# Autodesk Inventor assembly: Assembly
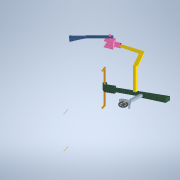
[picture p0: Inventor's stored thumbnail of the model, 180x180]
Saved by Autodesk Inventor 2021 (Build 250183000, 183)
## iProperties
Created: 2021-05-09
Part Number: Assembly
Document SubType Name: Assembly
Designer: Alsayaary
Author: Abdulrahman
## Documents named in this file (9)
- \\userAB\A\alsa0009\Desktop\seccuring mechanism\Assembly.iam
- \\userAB\A\alsa0009\Desktop\Securing mechanism paramatrised711\grip - C1-1.ipt
- \\userAB\A\alsa0009\Desktop\Securing mechanism paramatrised711\grip - C2-1.ipt
- \\userAB\A\alsa0009\Desktop\Securing mechanism paramatrised711\grip - C4-1.ipt
- \\userAB\A\alsa0009\Desktop\Securing mechanism paramatrised711\pin-1.ipt
- \\userAB\A\alsa0009\Desktop\Cad\sweep.ipt
- \\userAB\A\alsa0009\Desktop\Cad\wheel2.ipt
- \\userAB\A\alsa0009\Desktop\Securing mechanism paramatrised711\grip - Copy1-1.ipt
- \\userAB\A\alsa0009\Desktop\Cad\handle.ipt
## Components (8 placed, 8 different names)
1. grip - C1-1:1 — Mate:1, Mate:2, Flush:1, Mate:3, Flush:2, Mate:4, Mate:5, Mate:7, Mate:8, Flush:3, Mate:14, Transitional:1
2. grip - C2-1:1 — Mate:5, Mate:7, Mate:8, Flush:3, Mate:16, Mate:17, Mate:19
3. grip - C4-1:1 — Mate:3, Flush:2, Mate:4, Mate:15
4. sweep:1 — Mate:9, Mate:10, Transitional:1
5. wheel2:1 — Mate:15, Angle:3
6. pin-1:2 — Mate:16, Mate:18
7. grip - Copy1-1:1 — Mate:17, Mate:18, Mate:19, Mate:20, Mate:21
8. handle:1 — Mate:20, Mate:21
## Relationships (28: Mate 19, Flush 4, Angle 3, Symmetry 1, Transitional 1)
- Mate:1: grip - C1-1:1
- Mate:2: grip - C1-1:1
- Flush:1: grip - C1-1:1
- Mate:3: grip - C1-1:1 ↔ grip - C4-1:1
- Flush:2 (6.27 mm): grip - C1-1:1 ↔ grip - C4-1:1
- Mate:4 (231.798 mm): grip - C1-1:1 ↔ grip - C4-1:1
- Mate:5: grip - C1-1:1 ↔ grip - C2-1:1
- Mate:7: grip - C1-1:1 ↔ grip - C2-1:1
- Mate:8 (313.691 mm): grip - C1-1:1 ↔ grip - C2-1:1
- Flush:3: grip - C1-1:1 ↔ grip - C2-1:1
- Mate:9: sweep:1
- Mate:10: sweep:1
- Mate:11
- Angle:1 (0 deg)
- Mate:12
- Angle:2 (0 deg)
- Symmetry:1
- Flush:4
- Mate:14: grip - C1-1:1
- Mate:15: grip - C4-1:1 ↔ wheel2:1
- Angle:3 (0 deg): wheel2:1
- Mate:16: grip - C2-1:1 ↔ pin-1:2
- Transitional:1: grip - C1-1:1 ↔ sweep:1
- Mate:17: grip - C2-1:1 ↔ grip - Copy1-1:1
- Mate:18: pin-1:2 ↔ grip - Copy1-1:1
- Mate:19 (2 mm): grip - C2-1:1 ↔ grip - Copy1-1:1
- Mate:20: grip - Copy1-1:1 ↔ handle:1
- Mate:21 (5 mm): grip - Copy1-1:1 ↔ handle:1
